# Autodesk Inventor assembly: ASY NVPH-200 shredder shaft full
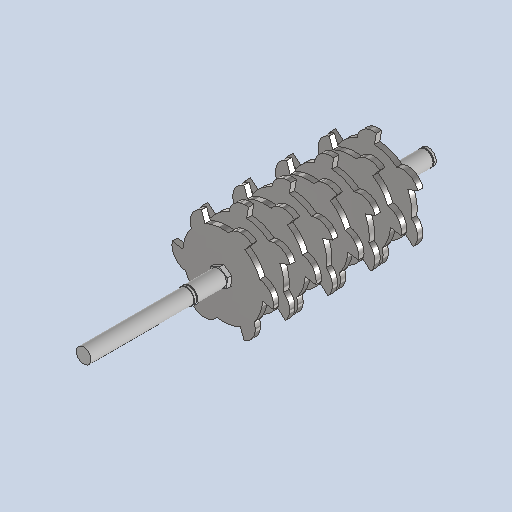
[picture p0: Inventor's stored thumbnail of the model, 512x512]
Saved by Autodesk Inventor 2025 (Build 290162010, 162A)
## iProperties
Created: 2024-12-05
Part Number: ASY NVPH-200 shredder shaft full
Document SubType Name: Assembly
Designer: user
Author: user
## Documents named in this file (4)
- C:\Users\DELL\YandexDisk-badmisterfox\домашниий пк\Inventor\NDM-VOS_powder_hopper\ASY NVPH-200 shredder shaft full.iam
- C:\Users\DELL\YandexDisk-badmisterfox\домашниий пк\Inventor\NDM-VOS_powder_hopper\NVPH-201 shredder shaft.ipt
- C:\Users\DELL\YandexDisk-badmisterfox\домашниий пк\Inventor\NDM-VOS_powder_hopper\NVPH-202 shredder cutter blade.ipt
- C:\Users\DELL\YandexDisk-badmisterfox\домашниий пк\Inventor\NDM-VOS_powder_hopper\NVPH-203 shredder cutter blade 3.ipt
## Components (9 placed, 3 different names)
1. NVPH-201 shredder shaft:1 — Rigid:1
2. NVPH-202 shredder cutter blade:1 — Rigid:1
3. NVPH-203 shredder cutter blade 3:1
4. NVPH-203 shredder cutter blade 3:2
5. NVPH-202 shredder cutter blade:2
6. NVPH-203 shredder cutter blade 3:3
7. NVPH-202 shredder cutter blade:3
8. NVPH-203 shredder cutter blade 3:4
9. NVPH-202 shredder cutter blade:4
## Component patterns: (4 elements, first: NVPH-202 shredder cutter blade:1 + NVPH-203 shredder cutter blade 3:1)
## Relationships (2: WeldJoint 2)
- Rigid:1 [WeldJoint] (8 mm): NVPH-201 shredder shaft:1 ↔ NVPH-202 shredder cutter blade:1
- [WeldJoint] (-40 mm): NVPH-202 shredder cutter blade:1 ↔ NVPH-203 shredder cutter blade 3:1
